# Autodesk Inventor assembly: AssyClimber
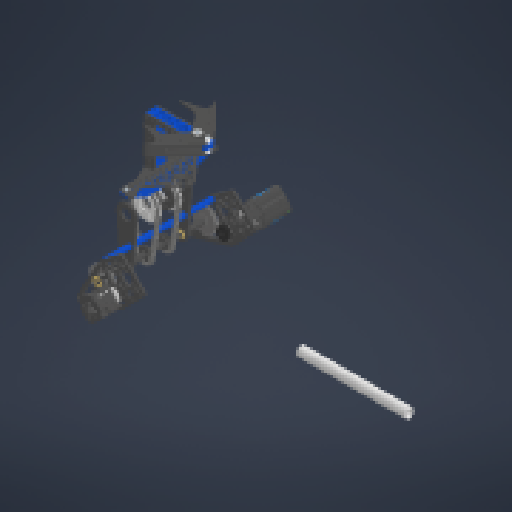
[picture p0: Inventor's stored thumbnail of the model, 512x512]
Saved by Autodesk Inventor 2024.3 (Build 283343000, 343)
## iProperties
Created: 2025-03-19
Part Number: AssyClimber
Document SubType Name: Assembly
Designer: jings
Author: jings
## Documents named in this file (7)
- C:\Users\jings\OneDrive\Desktop\FRC 5885\2025-Poseidon-Mechanical\climber\AssyClimber.iam
- C:\Users\jings\OneDrive\Desktop\FRC 5885\2025-Poseidon-Mechanical\climber\ClimberBottomBrace.ipt
- C:\Users\jings\OneDrive\Desktop\FRC 5885\2025-Poseidon-Mechanical\climber\ClimberFrame.ipt
- C:\Users\jings\OneDrive\Desktop\FRC 5885\2025-Poseidon-Mechanical\climber\ClimberHook1.ipt
- C:\Users\jings\OneDrive\Desktop\FRC 5885\2025-Poseidon-Mechanical\climber\ClimberHook2.ipt
- C:\Users\jings\OneDrive\Desktop\FRC 5885\2025-Poseidon-Mechanical\climber\ClimberAxel.ipt
- C:\Users\jings\Downloads\ClimberDriving\ClimberDriver\ClimberDriver.ipt
## Components (6 placed, 6 different names)
1. ClimberDriver:1 — Insert:6, Insert:7, Angle:3, Tangent:1
2. ClimberAxel:1 — Insert:7
3. ClimberBottomBrace:1 — Insert:3, Insert:4
4. ClimberFrame:1 — Insert:1, Insert:2, Insert:3, Insert:4, Insert:6
5. ClimberHook1:1 — Insert:1
6. ClimberHook2:1 — Insert:2
## Relationships (8: Insert 6, Angle 1, Tangent 1)
- Insert:1: ClimberFrame:1 ↔ ClimberHook1:1
- Insert:2: ClimberFrame:1 ↔ ClimberHook2:1
- Insert:3: ClimberBottomBrace:1 ↔ ClimberFrame:1
- Insert:4: ClimberBottomBrace:1 ↔ ClimberFrame:1
- Insert:6: ClimberDriver:1 ↔ ClimberFrame:1
- Insert:7 (-67.31 mm): ClimberDriver:1 ↔ ClimberAxel:1
- Angle:3 (-5 deg): ClimberDriver:1
- Tangent:1: ClimberDriver:1
